# Autodesk Inventor assembly: Z belt Sub
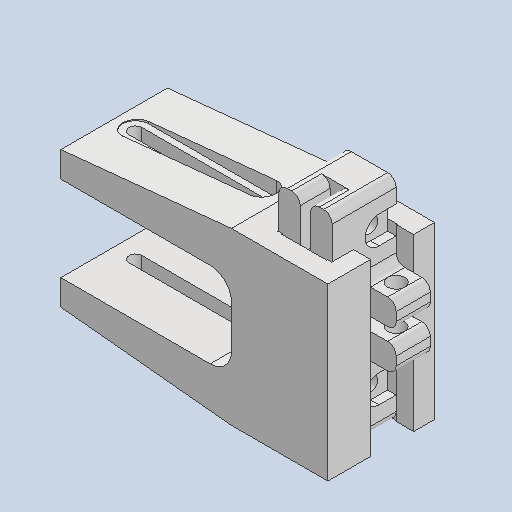
[picture p0: Inventor's stored thumbnail of the model, 512x512]
Saved by Autodesk Inventor 2022 (Build 260153000, 153)
## iProperties
Created: 2022-02-24
Part Number: Z belt Sub
Document SubType Name: Assembly
Designer: Nicoli
Author: Nicoli
## Documents named in this file (4)
- Y:\Projects\Bibble0\SubAsm\Z belt Sub.iam
- Y:\Projects\Bibble0\3D printed\Z Axis\Z Belt Clip.ipt
- Y:\Projects\Bibble0\3D printed\Z Axis\Z Belt Housing.ipt
- Y:\Projects\Bibble0\3D printed\Z Axis\Z Belt Tensioner - Mirror.ipt
## Components (3 placed, 3 different names)
1. Z Belt Clip:1 — Insert:1, Insert:2, Mate:3
2. Z Belt Housing:1 — Mate:2, Insert:1, Mate:3
3. Z Belt Tensioner - Mirror:1 — Mate:2, Insert:2
## Relationships (4: Mate 2, Insert 2)
- Mate:2: Z Belt Housing:1 ↔ Z Belt Tensioner - Mirror:1
- Insert:1: Z Belt Clip:1 ↔ Z Belt Housing:1
- Insert:2 (3 mm): Z Belt Clip:1 ↔ Z Belt Tensioner - Mirror:1
- Mate:3: Z Belt Clip:1 ↔ Z Belt Housing:1
